# Autodesk Inventor assembly: Klick-00_Xol_D2F_PCB _1__MIR_MIR
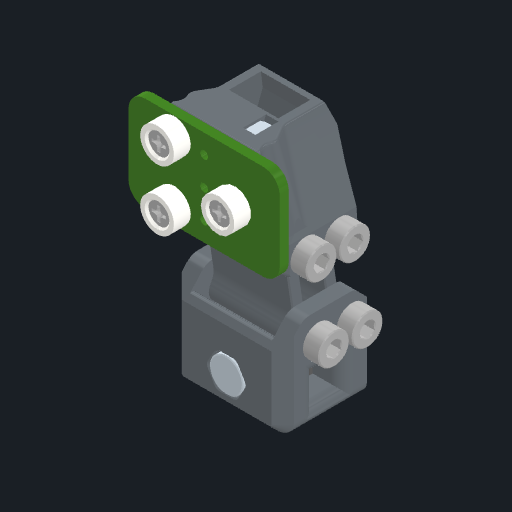
[picture p0: Inventor's stored thumbnail of the model, 512x512]
Saved by Autodesk Inventor 2024.3 (Build 283343010, 343A)
## iProperties
Created: 2024-12-01
Part Number: Klick-00_Xol_D2F_PCB _1__MIR_MIR
Document SubType Name: Assembly
Designer: MFil
Author: MFil
## Documents named in this file (11)
- C:\ROBOTYKA\myVORON-tridex\Hotend carriges\parts\Klicky-00 - RC2 Assemblies\Klicky-00 - RC2 Assemblies\Klick-00_Xol_D2F_PCB _1__MIR_MIR.iam
- C:\ROBOTYKA\myVORON-tridex\Hotend carriges\parts\Klicky-00 - RC2 Assemblies\Klicky-00 - RC2 Assemblies\Magnet [6x3]_MIR_MIR.ipt
- C:\ROBOTYKA\myVORON-tridex\Hotend carriges\parts\Klicky-00 - RC2 Assemblies\Klicky-00 - RC2 Assemblies\Klicky-00_PCB_Klicky_Rear_MIR_MIR.ipt
- C:\ROBOTYKA\myVORON-tridex\Hotend carriges\parts\Klicky-00 - RC2 Assemblies\Klicky-00 - RC2 Assemblies\Klicky-00_Xol_PCB_Swingarm_Upper_MIR_MIR.ipt
- C:\ROBOTYKA\myVORON-tridex\Hotend carriges\parts\Klicky-00 - RC2 Assemblies\Klicky-00 - RC2 Assemblies\D2F_ACTUATOR_MIR_MIR.ipt
- C:\ROBOTYKA\myVORON-tridex\Hotend carriges\parts\Klicky-00 - RC2 Assemblies\Klicky-00 - RC2 Assemblies\M2x10 FHCS self tapping screw_MIR_MIR.ipt
- C:\ROBOTYKA\myVORON-tridex\Hotend carriges\parts\Klicky-00 - RC2 Assemblies\Klicky-00 - RC2 Assemblies\Klicky-00_Xol_PCB_Swingarm_Lower_MIR_MIR.ipt
- C:\ROBOTYKA\myVORON-tridex\Hotend carriges\parts\Klicky-00 - RC2 Assemblies\Klicky-00 - RC2 Assemblies\M3x20 SHCS_MIR_MIR.ipt
- C:\ROBOTYKA\myVORON-tridex\Hotend carriges\parts\Klicky-00 - RC2 Assemblies\Klicky-00 - RC2 Assemblies\D2F_BASE_MIR_MIR.ipt
- C:\ROBOTYKA\myVORON-tridex\Hotend carriges\parts\Klicky-00 - RC2 Assemblies\Klicky-00 - RC2 Assemblies\Klicky-00_Xol_D2F_Front_MIR_MIR.ipt
- C:\ROBOTYKA\myVORON-tridex\Hotend carriges\parts\Klicky-00 - RC2 Assemblies\Klicky-00 - RC2 Assemblies\PCB-Klicky_Probe-side _1_ (2)_MIR_MIR.iam
## Components (17 placed, 10 different names)
1. Magnet [6x3]_MIR_MIR:1 — Mate:17, Mate:18
2. Klicky-00_PCB_Klicky_Rear_MIR_MIR:1 — Mate:13, Mate:15, Mate:7, Mate:8, Mate:12, Mate:14, Mate:16, Mate:11, Flush:6, Mate:1, Mate:2, Mate:3, Mate:4, Mate:5, Mate:6
3. Klicky-00_Xol_PCB_Swingarm_Upper_MIR_MIR:1 — Mate:13, Mate:15, Flush:1, Mate:19, Mate:20
4. D2F_ACTUATOR_MIR_MIR:1 — Mate:29, Mate:30, Mate:31
5. Magnet [6x3]_MIR_MIR:2 — Mate:9, Mate:10
6. Magnet [6x3]_MIR_MIR:3 — Mate:7, Mate:8
7. M2x10 FHCS self tapping screw_MIR_MIR:1 — Flush:4, Mate:27, Flush:5
8. Klicky-00_Xol_PCB_Swingarm_Lower_MIR_MIR:1 — Mate:9, Mate:10, Mate:12, Flush:1, Mate:21
9. M3x20 SHCS_MIR_MIR:1 — Mate:14, Mate:16, Flush:2
10. M3x20 SHCS_MIR_MIR:2 — Mate:11, Flush:2
11. D2F_BASE_MIR_MIR:1 — Mate:29, Mate:30, Mate:31, Mate:25, Mate:26, Mate:32
12. M3x20 SHCS_MIR_MIR:3 — Mate:23, Flush:3
13. M2x10 FHCS self tapping screw_MIR_MIR:2 — Flush:4, Mate:28
14. Klicky-00_Xol_D2F_Front_MIR_MIR:1 — Mate:17, Mate:18, Mate:19, Mate:20, Mate:21, Mate:23, Mate:25, Mate:26, Mate:27, Mate:28, Flush:5, Mate:32, Flush:6, Mate:22, Mate:24, Flush:7
15. M3x20 SHCS_MIR_MIR:4 — Mate:22, Flush:3, Mate:24
16. PCB-Klicky_Probe-side _1_ (2)_MIR_MIR:1 [sub-assembly] — Flush:7, Mate:1, Mate:2, Mate:3, Mate:4
17. Magnet [6x3]_MIR_MIR:4 — Mate:5, Mate:6
## Relationships (39: Mate 32, Flush 7)
- Mate:13: Klicky-00_PCB_Klicky_Rear_MIR_MIR:1 ↔ Klicky-00_Xol_PCB_Swingarm_Upper_MIR_MIR:1
- Mate:15 (0.1 mm): Klicky-00_PCB_Klicky_Rear_MIR_MIR:1 ↔ Klicky-00_Xol_PCB_Swingarm_Upper_MIR_MIR:1
- Mate:7: Klicky-00_PCB_Klicky_Rear_MIR_MIR:1 ↔ Magnet [6x3]_MIR_MIR:3
- Mate:8: Klicky-00_PCB_Klicky_Rear_MIR_MIR:1 ↔ Magnet [6x3]_MIR_MIR:3
- Mate:9: Magnet [6x3]_MIR_MIR:2 ↔ Klicky-00_Xol_PCB_Swingarm_Lower_MIR_MIR:1
- Mate:10: Magnet [6x3]_MIR_MIR:2 ↔ Klicky-00_Xol_PCB_Swingarm_Lower_MIR_MIR:1
- Mate:12: Klicky-00_PCB_Klicky_Rear_MIR_MIR:1 ↔ Klicky-00_Xol_PCB_Swingarm_Lower_MIR_MIR:1
- Flush:1: Klicky-00_Xol_PCB_Swingarm_Upper_MIR_MIR:1 ↔ Klicky-00_Xol_PCB_Swingarm_Lower_MIR_MIR:1
- Mate:14: Klicky-00_PCB_Klicky_Rear_MIR_MIR:1 ↔ M3x20 SHCS_MIR_MIR:1
- Mate:16: Klicky-00_PCB_Klicky_Rear_MIR_MIR:1 ↔ M3x20 SHCS_MIR_MIR:1
- Mate:11: Klicky-00_PCB_Klicky_Rear_MIR_MIR:1 ↔ M3x20 SHCS_MIR_MIR:2
- Flush:2: M3x20 SHCS_MIR_MIR:1 ↔ M3x20 SHCS_MIR_MIR:2
- Mate:29: D2F_ACTUATOR_MIR_MIR:1 ↔ D2F_BASE_MIR_MIR:1
- Mate:30: D2F_ACTUATOR_MIR_MIR:1 ↔ D2F_BASE_MIR_MIR:1
- Mate:31: D2F_ACTUATOR_MIR_MIR:1 ↔ D2F_BASE_MIR_MIR:1
- Flush:4: M2x10 FHCS self tapping screw_MIR_MIR:1 ↔ M2x10 FHCS self tapping screw_MIR_MIR:2
- Mate:17: Magnet [6x3]_MIR_MIR:1 ↔ Klicky-00_Xol_D2F_Front_MIR_MIR:1
- Mate:18: Magnet [6x3]_MIR_MIR:1 ↔ Klicky-00_Xol_D2F_Front_MIR_MIR:1
- Mate:19 (0.1 mm): Klicky-00_Xol_PCB_Swingarm_Upper_MIR_MIR:1 ↔ Klicky-00_Xol_D2F_Front_MIR_MIR:1
- Mate:20: Klicky-00_Xol_PCB_Swingarm_Upper_MIR_MIR:1 ↔ Klicky-00_Xol_D2F_Front_MIR_MIR:1
- Mate:21: Klicky-00_Xol_PCB_Swingarm_Lower_MIR_MIR:1 ↔ Klicky-00_Xol_D2F_Front_MIR_MIR:1
- Mate:23: M3x20 SHCS_MIR_MIR:3 ↔ Klicky-00_Xol_D2F_Front_MIR_MIR:1
- Mate:25: D2F_BASE_MIR_MIR:1 ↔ Klicky-00_Xol_D2F_Front_MIR_MIR:1
- Mate:26: D2F_BASE_MIR_MIR:1 ↔ Klicky-00_Xol_D2F_Front_MIR_MIR:1
- Mate:27: M2x10 FHCS self tapping screw_MIR_MIR:1 ↔ Klicky-00_Xol_D2F_Front_MIR_MIR:1
- Mate:28: M2x10 FHCS self tapping screw_MIR_MIR:2 ↔ Klicky-00_Xol_D2F_Front_MIR_MIR:1
- Flush:5: M2x10 FHCS self tapping screw_MIR_MIR:1 ↔ Klicky-00_Xol_D2F_Front_MIR_MIR:1
- Mate:32 (0.15 mm): D2F_BASE_MIR_MIR:1 ↔ Klicky-00_Xol_D2F_Front_MIR_MIR:1
- Flush:6: Klicky-00_PCB_Klicky_Rear_MIR_MIR:1 ↔ Klicky-00_Xol_D2F_Front_MIR_MIR:1
- Mate:22: Klicky-00_Xol_D2F_Front_MIR_MIR:1 ↔ M3x20 SHCS_MIR_MIR:4
- Flush:3: M3x20 SHCS_MIR_MIR:3 ↔ M3x20 SHCS_MIR_MIR:4
- Mate:24: Klicky-00_Xol_D2F_Front_MIR_MIR:1 ↔ M3x20 SHCS_MIR_MIR:4
- Flush:7 (4 mm): Klicky-00_Xol_D2F_Front_MIR_MIR:1 ↔ PCB-Klicky_Probe-side _1_ (2)_MIR_MIR:1
- Mate:1: Klicky-00_PCB_Klicky_Rear_MIR_MIR:1 ↔ PCB-Klicky_Probe-side _1_ (2)_MIR_MIR:1
- Mate:2: Klicky-00_PCB_Klicky_Rear_MIR_MIR:1 ↔ PCB-Klicky_Probe-side _1_ (2)_MIR_MIR:1
- Mate:3: Klicky-00_PCB_Klicky_Rear_MIR_MIR:1 ↔ PCB-Klicky_Probe-side _1_ (2)_MIR_MIR:1
- Mate:4: Klicky-00_PCB_Klicky_Rear_MIR_MIR:1 ↔ PCB-Klicky_Probe-side _1_ (2)_MIR_MIR:1
- Mate:5: Klicky-00_PCB_Klicky_Rear_MIR_MIR:1 ↔ Magnet [6x3]_MIR_MIR:4
- Mate:6: Klicky-00_PCB_Klicky_Rear_MIR_MIR:1 ↔ Magnet [6x3]_MIR_MIR:4
